# Autodesk Inventor assembly: 6 Axis Manipulator Axis 5 and 6 Assembly
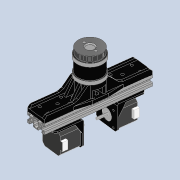
[picture p0: Inventor's stored thumbnail of the model, 180x180]
Saved by Autodesk Inventor 2022 (Build 260153000, 153)
## iProperties
Created: 2021-12-24
Part Number: 6 Axis Manipulator Axis 5 and 6 Assembly
Document SubType Name: Assembly
Designer: Coy
Author: Coy
## Documents named in this file (9)
- H:\3D Files\Project 3D Models\Breakfast Maker 2000\Assemblys\6 Axis Manipulator Axis 5 and 6 Assembly.iam
- H:\3D Files\Project 3D Models\Breakfast Maker 2000\Nema 17 Stepper Motor Mounting Bracket.ipt
- H:\3D Files\Project 3D Models\Breakfast Maker 2000\Motors\Nema 17 Stepper Motor 37mm.ipt
- H:\3D Files\Project 3D Models\Breakfast Maker 2000\90 deg Shelf 4 Hole Bracket.ipt
- H:\3D Files\Project 3D Models\Breakfast Maker 2000\Aluminum Extrusion\2040\2040x200 silver profile.ipt
- H:\3D Files\Project 3D Models\Breakfast Maker 2000\3D Printed Parts\Axis 4 Male Bearing Connector Bracket.ipt
- H:\3D Files\Project 3D Models\Breakfast Maker 2000\Bearings\40mm ID 52mm OD 7mm Deep Roller Bearing (2021_08_15 23_37_01 UTC).ipt
- H:\3D Files\Project 3D Models\Breakfast Maker 2000\3D Printed Parts\Axis 4 Bearing 25mm Spacer.ipt
- H:\3D Files\Project 3D Models\Breakfast Maker 2000\Pullys\GT2 72 Tooth Timing Belt Pulley.ipt
## Components (12 placed, 8 different names)
1. Nema 17 Stepper Motor Mounting Bracket:1 — Mate:14, Angle:3, Mate:15, Mate:41, Mate:43, Flush:25
2. Nema 17 Stepper Motor Mounting Bracket:2 — Mate:12, Angle:2, Mate:13, Mate:42, Mate:43, Flush:25, Flush:26, Flush:27
3. Nema 17 Stepper Motor 37mm:1 — Mate:12, Angle:2, Mate:13
4. Nema 17 Stepper Motor 37mm:2 — Mate:14, Angle:3, Mate:15
5. 2040x200 silver profile:1 — Mate:25, Flush:23, Flush:24, Mate:41, Mate:42, Flush:26, Flush:27
6. Axis 4 Male Bearing Connector Bracket:1 — Mate:25, Flush:23, Flush:24, Mate:26, Mate:27, Mate:28, Mate:29, Mate:32, Mate:33, Mate:34, Mate:35, Mate:36, Mate:37, Mate:38, Mate:39, Mate:40
7. 40mm ID 52mm OD 7mm Deep Roller Bearing (2021_08_15 23_37_01 UTC):1 — Mate:28, Mate:31
8. 40mm ID 52mm OD 7mm Deep Roller Bearing (2021_08_15 23_37_01 UTC):2 — Mate:26, Mate:27, Mate:30
9. Axis 4 Bearing 25mm Spacer:1 — Mate:29, Mate:30, Mate:31
10. GT2 72 Tooth Timing Belt Pulley:1 — Mate:32, Mate:33, Mate:34
11. 90 deg Shelf 4 Hole Bracket:9 — Mate:35, Mate:36, Mate:37
12. 90 deg Shelf 4 Hole Bracket:10 — Mate:38, Mate:39, Mate:40
## Relationships (30: Mate 23, Flush 5, Angle 2)
- Mate:12: Nema 17 Stepper Motor Mounting Bracket:2 ↔ Nema 17 Stepper Motor 37mm:1
- Angle:2 (0 deg): Nema 17 Stepper Motor Mounting Bracket:2 ↔ Nema 17 Stepper Motor 37mm:1
- Mate:13: Nema 17 Stepper Motor Mounting Bracket:2 ↔ Nema 17 Stepper Motor 37mm:1
- Mate:14: Nema 17 Stepper Motor Mounting Bracket:1 ↔ Nema 17 Stepper Motor 37mm:2
- Angle:3 (0 deg): Nema 17 Stepper Motor Mounting Bracket:1 ↔ Nema 17 Stepper Motor 37mm:2
- Mate:15: Nema 17 Stepper Motor Mounting Bracket:1 ↔ Nema 17 Stepper Motor 37mm:2
- Mate:25: 2040x200 silver profile:1 ↔ Axis 4 Male Bearing Connector Bracket:1
- Flush:23: 2040x200 silver profile:1 ↔ Axis 4 Male Bearing Connector Bracket:1
- Flush:24: 2040x200 silver profile:1 ↔ Axis 4 Male Bearing Connector Bracket:1
- Mate:26: Axis 4 Male Bearing Connector Bracket:1 ↔ 40mm ID 52mm OD 7mm Deep Roller Bearing (2021_08_15 23_37_01 UTC):2
- Mate:27: Axis 4 Male Bearing Connector Bracket:1 ↔ 40mm ID 52mm OD 7mm Deep Roller Bearing (2021_08_15 23_37_01 UTC):2
- Mate:28: Axis 4 Male Bearing Connector Bracket:1 ↔ 40mm ID 52mm OD 7mm Deep Roller Bearing (2021_08_15 23_37_01 UTC):1
- Mate:29: Axis 4 Male Bearing Connector Bracket:1 ↔ Axis 4 Bearing 25mm Spacer:1
- Mate:30: 40mm ID 52mm OD 7mm Deep Roller Bearing (2021_08_15 23_37_01 UTC):2 ↔ Axis 4 Bearing 25mm Spacer:1
- Mate:31: 40mm ID 52mm OD 7mm Deep Roller Bearing (2021_08_15 23_37_01 UTC):1 ↔ Axis 4 Bearing 25mm Spacer:1
- Mate:32: Axis 4 Male Bearing Connector Bracket:1 ↔ GT2 72 Tooth Timing Belt Pulley:1
- Mate:33: Axis 4 Male Bearing Connector Bracket:1 ↔ GT2 72 Tooth Timing Belt Pulley:1
- Mate:34: Axis 4 Male Bearing Connector Bracket:1 ↔ GT2 72 Tooth Timing Belt Pulley:1
- Mate:35: Axis 4 Male Bearing Connector Bracket:1 ↔ 90 deg Shelf 4 Hole Bracket:9
- Mate:36: Axis 4 Male Bearing Connector Bracket:1 ↔ 90 deg Shelf 4 Hole Bracket:9
- Mate:37: Axis 4 Male Bearing Connector Bracket:1 ↔ 90 deg Shelf 4 Hole Bracket:9
- Mate:38: Axis 4 Male Bearing Connector Bracket:1 ↔ 90 deg Shelf 4 Hole Bracket:10
- Mate:39: Axis 4 Male Bearing Connector Bracket:1 ↔ 90 deg Shelf 4 Hole Bracket:10
- Mate:40: Axis 4 Male Bearing Connector Bracket:1 ↔ 90 deg Shelf 4 Hole Bracket:10
- Mate:41: Nema 17 Stepper Motor Mounting Bracket:1 ↔ 2040x200 silver profile:1
- Mate:42: Nema 17 Stepper Motor Mounting Bracket:2 ↔ 2040x200 silver profile:1
- Mate:43 (62 mm): Nema 17 Stepper Motor Mounting Bracket:1 ↔ Nema 17 Stepper Motor Mounting Bracket:2
- Flush:25: Nema 17 Stepper Motor Mounting Bracket:1 ↔ Nema 17 Stepper Motor Mounting Bracket:2
- Flush:26 (-5 mm): Nema 17 Stepper Motor Mounting Bracket:2 ↔ 2040x200 silver profile:1
- Flush:27 (15 mm): Nema 17 Stepper Motor Mounting Bracket:2 ↔ 2040x200 silver profile:1
